# Autodesk Inventor assembly: TCP_Final
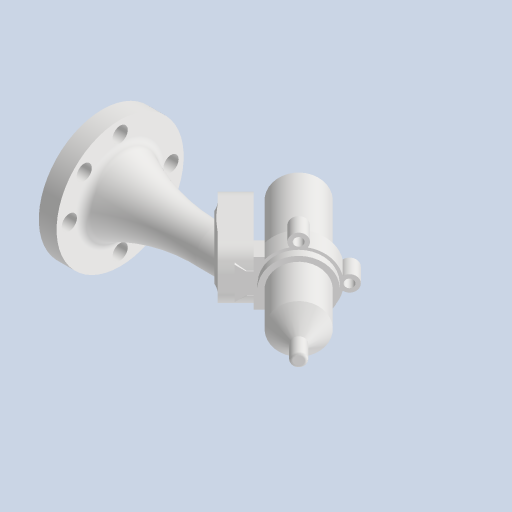
[picture p0: Inventor's stored thumbnail of the model, 512x512]
Saved by Autodesk Inventor 2024 (Build 280153000, 153)
## iProperties
Created: 2025-06-11
Part Number: TCP_Final
Document SubType Name: Assembly
Designer: ANDRES
Author: ANDRES
## Documents named in this file (5)
- C:\Users\ANDRES\Documents\Universidad\Robotica\Laboratorios\Laboratorio 2\TCP_Final.iam
- C:\Users\ANDRES\Documents\Universidad\Robotica\Laboratorios\Laboratorio 2\acople_v2.ipt
- C:\Users\ANDRES\Documents\Universidad\Robotica\Laboratorios\Laboratorio 2\Porta herramientas p1.ipt
- C:\Users\ANDRES\Documents\Universidad\Robotica\Laboratorios\Laboratorio 2\Porta herramientas p2.ipt
- C:\Users\ANDRES\Documents\Universidad\Robotica\Laboratorios\Laboratorio 2\Marcador_V2.ipt
## Components (4 placed, 4 different names)
1. acople_v2:1 — Coincidencia:4, Coincidencia:5, Coincidencia:6, Nivelación:1, Coincidencia:8, Coincidencia:9
2. Porta herramientas p1:1 — Coincidencia:1, Coincidencia:2, Coincidencia:3
3. Porta herramientas p2:1 — Coincidencia:1, Coincidencia:2, Coincidencia:3, Coincidencia:4, Coincidencia:5, Coincidencia:6
4. Marcador_V2:1 — Coincidencia:8, Coincidencia:9
## Relationships (9: Mate 8, Flush 1)
- Coincidencia:1 [Mate]: Porta herramientas p1:1 ↔ Porta herramientas p2:1
- Coincidencia:2 [Mate]: Porta herramientas p1:1 ↔ Porta herramientas p2:1
- Coincidencia:3 [Mate]: Porta herramientas p1:1 ↔ Porta herramientas p2:1
- Coincidencia:4 [Mate]: acople_v2:1 ↔ Porta herramientas p2:1
- Coincidencia:5 [Mate] (0.15 mm): acople_v2:1 ↔ Porta herramientas p2:1
- Coincidencia:6 [Mate] (0.1 mm): acople_v2:1 ↔ Porta herramientas p2:1
- Nivelación:1 [Flush] (8.6 mm): acople_v2:1
- Coincidencia:8 [Mate]: acople_v2:1 ↔ Marcador_V2:1
- Coincidencia:9 [Mate]: acople_v2:1 ↔ Marcador_V2:1
